# Autodesk Inventor assembly: 3.25 Omni AS, Circle_MIR3
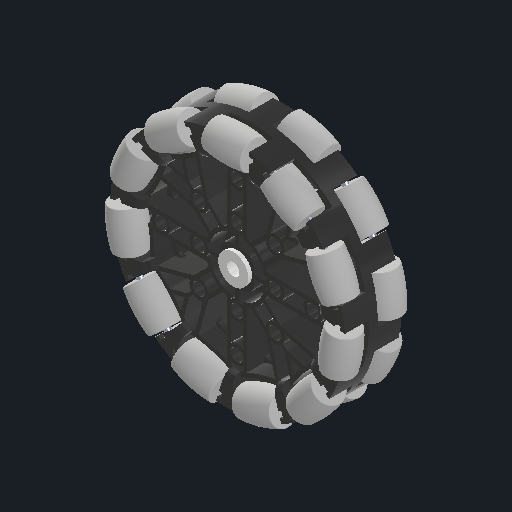
[picture p0: Inventor's stored thumbnail of the model, 512x512]
Saved by Autodesk Inventor 2024 (Build 280153000, 153)
## iProperties
Created: 2022-08-02
Part Number: 3.25 Omni AS, Circle_MIR3
Document SubType Name: Assembly
Designer: macbook
Author: ylu12
## Documents named in this file (3)
- \\Mac\Home\Desktop\code\1899V-VRC\Cad\Motion\Wheels\Omni Wheel\3.25 Omni AS, Circle_MIR3.iam
- \\Mac\Home\Desktop\code\1899V-VRC\Cad\Motion\Wheels\Reference Files\3.25 Omni Antistatic_MIR3.ipt
- \\Mac\Home\Desktop\code\1899V-VRC\Cad\Motion\Insert Circle_MIR4.ipt
## Components (3 placed, 2 different names)
1. 3.25 Omni Antistatic_MIR3:1 — Mate:12, Mate:11, Flush:6
2. Insert Circle_MIR4:1 — Angle:2, Mate:20, Flush:13, Flush:12, Flush:14
3. Insert Circle_MIR4:2 — Flush:13, Flush:12, Mate:19
## Relationships (9: Mate 4, Flush 4, Angle 1)
- Mate:12: 3.25 Omni Antistatic_MIR3:1
- Mate:11: 3.25 Omni Antistatic_MIR3:1
- Flush:6: 3.25 Omni Antistatic_MIR3:1
- Angle:2 (0 deg): Insert Circle_MIR4:1
- Mate:20: Insert Circle_MIR4:1
- Flush:13: Insert Circle_MIR4:1 ↔ Insert Circle_MIR4:2
- Flush:12: Insert Circle_MIR4:1 ↔ Insert Circle_MIR4:2
- Flush:14 [Mate] (6.35 mm): Insert Circle_MIR4:1
- Mate:19 [Flush] (6.35 mm): Insert Circle_MIR4:2
